# Autodesk Inventor assembly: RightDriveAssembly
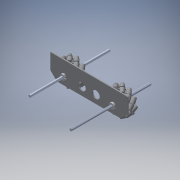
[picture p0: Inventor's stored thumbnail of the model, 180x180]
Saved by Autodesk Inventor 2017 (Build 210142000, 142)
## iProperties
Created: 2017-09-16
Part Number: RightDriveAssembly
Document SubType Name: Assembly
Designer: User
Author: User
## Documents named in this file (8)
- C:\Robotics\CAD\2017-18_CAD\RightDriveAssembly.iam
- C:\Robotics\CAD\2017-18_CAD\MecanumDriveTrainPlate17-18.ipt
- C:\Robotics\CAD\COTSParts\Vex\6inchMecanumRight217-2586-STEP\6inchMecanumRight217-2586.20121203.ipt
- C:\Robotics\CAD\COTSParts\Vex\HexBearings.5inchBore217-3875-STEP-20140818\HexBearings.5inchBore217-3875-STEP-20140818.ipt
- C:\Robotics\CAD\COTSParts\Vex\HexAxle.5inchOD217-3309-STEP\HexAxle.5inchOD18inchLength217-3309-STEP.ipt
- C:\Robotics\CAD\COTSParts\Vex\CollarClamp.5\am-1238+Collar+Clamp,+0.5''+Hex+Bore,+Aluminum.iam
- C:\Robotics\CAD\COTSParts\Vex\VersaHub.5inchBore217-4009-STEP-20140807\VersaHub.5inchBore217-4009-STEP-20140807.ipt
- C:\Robotics\CAD\COTSParts\Vex\HexSprocket.5inchBore\HexSprocket18t.5inchBore217-3488-STEP\HexSprocket18t.5inchBore217-3488-STEP.ipt
## Components (19 placed, 7 different names)
1. MecanumDriveTrainPlate17-18:1 — Mate:12, Mate:31, Mate:37, Mate:40, Mate:41
2. 6inchMecanumRight217-2586.20121203:1 — Mate:13, Mate:14, Mate:15, Mate:16, Mate:17, Mate:18
3. HexBearings.5inchBore217-3875-STEP-20140818:1 — Mate:3, Mate:4, Mate:5, Mate:41
4. HexAxle.5inchOD18inchLength217-3309-STEP:1 — Mate:32, Mate:33, Mate:35, Mate:36, Mate:38, Mate:39, Mate:55, Mate:57, Mate:59, Mate:60, Mate:62, Mate:63
5. HexAxle.5inchOD18inchLength217-3309-STEP:2 — Mate:1, Mate:2, Mate:4, Mate:5, Mate:10, Mate:11, Mate:26, Mate:27, Mate:45, Mate:46, Mate:48, Mate:49
6. HexBearings.5inchBore217-3875-STEP-20140818:2 — Mate:31, Mate:32, Mate:33, Mate:34, Mate:40
7. am-1238+Collar+Clamp,+0.5''+Hex+Bore,+Aluminum:1 [sub-assembly] — Mate:44, Mate:45, Mate:46, Mate:47
8. am-1238+Collar+Clamp,+0.5''+Hex+Bore,+Aluminum:2 [sub-assembly] — Mate:1, Mate:2, Mate:3
9. am-1238+Collar+Clamp,+0.5''+Hex+Bore,+Aluminum:3 [sub-assembly] — Mate:10, Mate:11, Mate:12, Mate:25
10. am-1238+Collar+Clamp,+0.5''+Hex+Bore,+Aluminum:4 [sub-assembly] — Mate:37, Mate:38, Mate:39, Mate:56
11. am-1238+Collar+Clamp,+0.5''+Hex+Bore,+Aluminum:5 [sub-assembly] — Mate:34, Mate:35, Mate:36
12. am-1238+Collar+Clamp,+0.5''+Hex+Bore,+Aluminum:6 [sub-assembly] — Mate:58, Mate:59, Mate:60, Mate:61
13. HexSprocket18t.5inchBore217-3488-STEP:1 — Mate:47, Mate:48, Mate:49
14. HexSprocket18t.5inchBore217-3488-STEP:2 — Mate:61, Mate:62, Mate:63
15. VersaHub.5inchBore217-4009-STEP-20140807:2 — Mate:13, Mate:14, Mate:15, Mate:25
16. VersaHub.5inchBore217-4009-STEP-20140807:4 — Mate:16, Mate:17, Mate:18, Mate:26, Mate:27, Mate:44
17. VersaHub.5inchBore217-4009-STEP-20140807:5 — Mate:53, Mate:54, Mate:56
18. VersaHub.5inchBore217-4009-STEP-20140807:6 — Mate:50, Mate:51, Mate:52, Mate:55, Mate:57, Mate:58
19. 6inchMecanumRight217-2586.20121203:2 — Mate:50, Mate:51, Mate:52, Mate:53, Mate:54
## Relationships (48: Mate 48)
- Mate:1: HexAxle.5inchOD18inchLength217-3309-STEP:2 ↔ am-1238+Collar+Clamp,+0.5''+Hex+Bore,+Aluminum:2
- Mate:2: HexAxle.5inchOD18inchLength217-3309-STEP:2 ↔ am-1238+Collar+Clamp,+0.5''+Hex+Bore,+Aluminum:2
- Mate:3: HexBearings.5inchBore217-3875-STEP-20140818:1 ↔ am-1238+Collar+Clamp,+0.5''+Hex+Bore,+Aluminum:2
- Mate:4: HexBearings.5inchBore217-3875-STEP-20140818:1 ↔ HexAxle.5inchOD18inchLength217-3309-STEP:2
- Mate:5: HexBearings.5inchBore217-3875-STEP-20140818:1 ↔ HexAxle.5inchOD18inchLength217-3309-STEP:2
- Mate:10: HexAxle.5inchOD18inchLength217-3309-STEP:2 ↔ am-1238+Collar+Clamp,+0.5''+Hex+Bore,+Aluminum:3
- Mate:11: HexAxle.5inchOD18inchLength217-3309-STEP:2 ↔ am-1238+Collar+Clamp,+0.5''+Hex+Bore,+Aluminum:3
- Mate:12 (3.175 mm): MecanumDriveTrainPlate17-18:1 ↔ am-1238+Collar+Clamp,+0.5''+Hex+Bore,+Aluminum:3
- Mate:13: 6inchMecanumRight217-2586.20121203:1 ↔ VersaHub.5inchBore217-4009-STEP-20140807:2
- Mate:14: 6inchMecanumRight217-2586.20121203:1 ↔ VersaHub.5inchBore217-4009-STEP-20140807:2
- Mate:15: 6inchMecanumRight217-2586.20121203:1 ↔ VersaHub.5inchBore217-4009-STEP-20140807:2
- Mate:16: 6inchMecanumRight217-2586.20121203:1 ↔ VersaHub.5inchBore217-4009-STEP-20140807:4
- Mate:17: 6inchMecanumRight217-2586.20121203:1 ↔ VersaHub.5inchBore217-4009-STEP-20140807:4
- Mate:18: 6inchMecanumRight217-2586.20121203:1 ↔ VersaHub.5inchBore217-4009-STEP-20140807:4
- Mate:25: am-1238+Collar+Clamp,+0.5''+Hex+Bore,+Aluminum:3 ↔ VersaHub.5inchBore217-4009-STEP-20140807:2
- Mate:26: HexAxle.5inchOD18inchLength217-3309-STEP:2 ↔ VersaHub.5inchBore217-4009-STEP-20140807:4
- Mate:27: HexAxle.5inchOD18inchLength217-3309-STEP:2 ↔ VersaHub.5inchBore217-4009-STEP-20140807:4
- Mate:31: MecanumDriveTrainPlate17-18:1 ↔ HexBearings.5inchBore217-3875-STEP-20140818:2
- Mate:32: HexAxle.5inchOD18inchLength217-3309-STEP:1 ↔ HexBearings.5inchBore217-3875-STEP-20140818:2
- Mate:33: HexAxle.5inchOD18inchLength217-3309-STEP:1 ↔ HexBearings.5inchBore217-3875-STEP-20140818:2
- Mate:34: HexBearings.5inchBore217-3875-STEP-20140818:2 ↔ am-1238+Collar+Clamp,+0.5''+Hex+Bore,+Aluminum:5
- Mate:35: HexAxle.5inchOD18inchLength217-3309-STEP:1 ↔ am-1238+Collar+Clamp,+0.5''+Hex+Bore,+Aluminum:5
- Mate:36: HexAxle.5inchOD18inchLength217-3309-STEP:1 ↔ am-1238+Collar+Clamp,+0.5''+Hex+Bore,+Aluminum:5
- Mate:37 (3.175 mm): MecanumDriveTrainPlate17-18:1 ↔ am-1238+Collar+Clamp,+0.5''+Hex+Bore,+Aluminum:4
- Mate:38: HexAxle.5inchOD18inchLength217-3309-STEP:1 ↔ am-1238+Collar+Clamp,+0.5''+Hex+Bore,+Aluminum:4
- Mate:39: HexAxle.5inchOD18inchLength217-3309-STEP:1 ↔ am-1238+Collar+Clamp,+0.5''+Hex+Bore,+Aluminum:4
- Mate:40: MecanumDriveTrainPlate17-18:1 ↔ HexBearings.5inchBore217-3875-STEP-20140818:2
- Mate:41: MecanumDriveTrainPlate17-18:1 ↔ HexBearings.5inchBore217-3875-STEP-20140818:1
- Mate:44: am-1238+Collar+Clamp,+0.5''+Hex+Bore,+Aluminum:1 ↔ VersaHub.5inchBore217-4009-STEP-20140807:4
- Mate:45: HexAxle.5inchOD18inchLength217-3309-STEP:2 ↔ am-1238+Collar+Clamp,+0.5''+Hex+Bore,+Aluminum:1
- Mate:46: HexAxle.5inchOD18inchLength217-3309-STEP:2 ↔ am-1238+Collar+Clamp,+0.5''+Hex+Bore,+Aluminum:1
- Mate:47: am-1238+Collar+Clamp,+0.5''+Hex+Bore,+Aluminum:1 ↔ HexSprocket18t.5inchBore217-3488-STEP:1
- Mate:48: HexAxle.5inchOD18inchLength217-3309-STEP:2 ↔ HexSprocket18t.5inchBore217-3488-STEP:1
- Mate:49: HexAxle.5inchOD18inchLength217-3309-STEP:2 ↔ HexSprocket18t.5inchBore217-3488-STEP:1
- Mate:50: VersaHub.5inchBore217-4009-STEP-20140807:6 ↔ 6inchMecanumRight217-2586.20121203:2
- Mate:51: VersaHub.5inchBore217-4009-STEP-20140807:6 ↔ 6inchMecanumRight217-2586.20121203:2
- Mate:52: VersaHub.5inchBore217-4009-STEP-20140807:6 ↔ 6inchMecanumRight217-2586.20121203:2
- Mate:53: VersaHub.5inchBore217-4009-STEP-20140807:5 ↔ 6inchMecanumRight217-2586.20121203:2
- Mate:54: VersaHub.5inchBore217-4009-STEP-20140807:5 ↔ 6inchMecanumRight217-2586.20121203:2
- Mate:55: HexAxle.5inchOD18inchLength217-3309-STEP:1 ↔ VersaHub.5inchBore217-4009-STEP-20140807:6
- Mate:56: am-1238+Collar+Clamp,+0.5''+Hex+Bore,+Aluminum:4 ↔ VersaHub.5inchBore217-4009-STEP-20140807:5
- Mate:57: HexAxle.5inchOD18inchLength217-3309-STEP:1 ↔ VersaHub.5inchBore217-4009-STEP-20140807:6
- Mate:58: am-1238+Collar+Clamp,+0.5''+Hex+Bore,+Aluminum:6 ↔ VersaHub.5inchBore217-4009-STEP-20140807:6
- Mate:59: HexAxle.5inchOD18inchLength217-3309-STEP:1 ↔ am-1238+Collar+Clamp,+0.5''+Hex+Bore,+Aluminum:6
- Mate:60: HexAxle.5inchOD18inchLength217-3309-STEP:1 ↔ am-1238+Collar+Clamp,+0.5''+Hex+Bore,+Aluminum:6
- Mate:61: am-1238+Collar+Clamp,+0.5''+Hex+Bore,+Aluminum:6 ↔ HexSprocket18t.5inchBore217-3488-STEP:2
- Mate:62: HexAxle.5inchOD18inchLength217-3309-STEP:1 ↔ HexSprocket18t.5inchBore217-3488-STEP:2
- Mate:63: HexAxle.5inchOD18inchLength217-3309-STEP:1 ↔ HexSprocket18t.5inchBore217-3488-STEP:2
